# Autodesk Inventor assembly: Assembly1
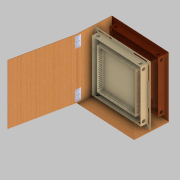
[picture p0: Inventor's stored thumbnail of the model, 180x180]
Saved by Autodesk Inventor 2020 (Build 240168000, 168)
## iProperties
Created: 2020-05-03
Part Number: Assembly1
Document SubType Name: Assembly
Designer: galaxy
Author: galaxy
## Documents named in this file (7)
- C:\Users\LENOVO\Desktop\Graduation Project\Fish Farming Unit\Control Box\Assembly1.iam
- C:\Users\LENOVO\Desktop\Graduation Project\Fish Farming Unit\Control Box\backside.ipt
- C:\Users\LENOVO\Desktop\Graduation Project\Fish Farming Unit\Control Box\down_cover.ipt
- C:\Users\LENOVO\Desktop\Graduation Project\Fish Farming Unit\Control Box\rightside.ipt
- C:\Users\LENOVO\Desktop\Graduation Project\Fish Farming Unit\Control Box\leftside_hinge.iam
- C:\Users\LENOVO\Desktop\Graduation Project\Fish Farming Unit\Control Box\middle.ipt
- C:\Users\LENOVO\Desktop\Graduation Project\Fish Farming Unit\Control Box\front_hings.iam
## Components (6 placed, 6 different names)
1. backside:1 — Mate:3, Mate:4, Mate:5, Mate:6, Mate:8
2. rightside:1 — Mate:3, Mate:4, Mate:7
3. leftside_hinge:1 [sub-assembly] — Mate:5, Mate:6, Insert:3
4. down_cover:2 — Mate:7, Mate:8, Insert:1, Insert:2
5. middle:1 — Insert:1, Insert:2
6. front_hings:1 [sub-assembly] — Insert:3
## Relationships (9: Mate 6, Insert 3)
- Mate:3: backside:1 ↔ rightside:1
- Mate:4: backside:1 ↔ rightside:1
- Mate:5: backside:1 ↔ leftside_hinge:1
- Mate:6: backside:1 ↔ leftside_hinge:1
- Mate:7: rightside:1 ↔ down_cover:2
- Mate:8: backside:1 ↔ down_cover:2
- Insert:1: down_cover:2 ↔ middle:1
- Insert:2: down_cover:2 ↔ middle:1
- Insert:3: leftside_hinge:1 ↔ front_hings:1
